# Autodesk Inventor assembly: drivepulleyAssembly
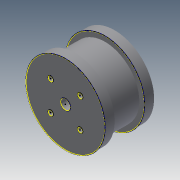
[picture p0: Inventor's stored thumbnail of the model, 180x180]
Saved by Autodesk Inventor 2015 (Build 190159000, 159)
## iProperties
Created: 2014-09-01
Part Number: drivepulleyAssembly
Document SubType Name: Assembly
Designer: shohei
Author: shohei
## Documents named in this file (3)
- C:\Users\shohei\Documents\Inventor\FufuPounderGeared\drivepulleyAssembly.iam
- C:\Users\shohei\Documents\Inventor\FufuPounderGeared\drivepulleyMiddle.ipt
- C:\Users\shohei\Documents\Inventor\FufuPounderGeared\drivepullySide.ipt
## Components (3 placed, 2 different names)
1. drivepulleyMiddle:1 — Mate:1, Mate:2
2. drivepullySide:1 — Mate:2
3. drivepullySide:2 — Mate:1
## Relationships (2: Mate 2)
- Mate:1: drivepulleyMiddle:1 ↔ drivepullySide:2
- Mate:2: drivepulleyMiddle:1 ↔ drivepullySide:1
